# Autodesk Inventor assembly: 6P Sprocket
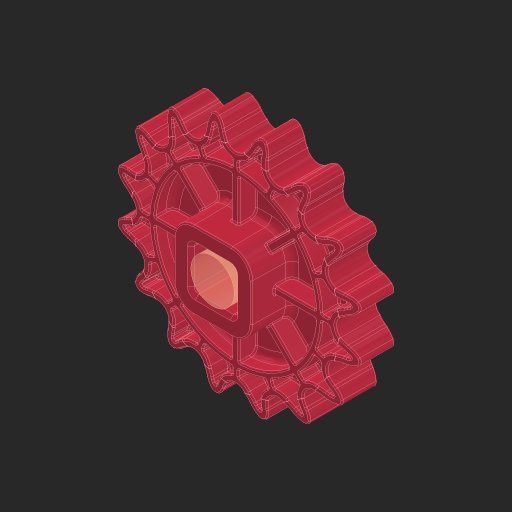
[picture p0: Inventor's stored thumbnail of the model, 512x512]
Saved by Autodesk Inventor 2023 (Build 270158000, 158)
## iProperties
Created: 2022-08-02
Part Number: 6P Sprocket
Document SubType Name: Assembly
Designer: ylu12
Author: ylu12
## Documents named in this file (3)
- C:\Users\ylu12\Documents\GitHub\VEX-CAD-Inventor\Motion\Sprockets\6P Sprocket\6P 16T Sprocket, No Insert.iam
- C:\Users\ylu12\Documents\GitHub\VEX-CAD-Inventor\Motion\Sprockets\Reference Files\6P 16T Sprocket.ipt
- C:\Users\ylu12\Documents\GitHub\VEX-CAD-Inventor\Motion\Sprockets\6P Sprocket.iam
## Components (1 placed, 1 different names)
1. 16T — Flush:4, Mate:7, Mate:8
## Relationships (3: Mate 2, Flush 1)
- Flush:4: 16T
- Mate:7: 16T
- Mate:8: 16T
